# Autodesk Inventor assembly: 174376 FNC-32
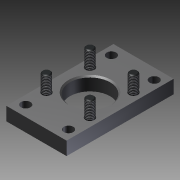
[picture p0: Inventor's stored thumbnail of the model, 180x180]
Saved by Autodesk Inventor 2011 SP1 (Build 150282100, 282)
## iProperties
Created: 2018-05-26
Part Number: 174376 FNC-32
Catalog Web Link: www.cadenas.de
Description: FNC-Flange mounting
Vendor: FESTO
Document SubType Name: Assembly
Designer: psAdmin
Manufacturer: FESTO
Mass: 221 g
Category: PARTsolutions
Company: FESTO
Title: 174376 FNC-32
Author: Cadenas PARTsolutions
Comments: Flange mounting
PSOL_IDENT_0: {$CADENAS_DATA\23d-libs\festo\parts\f\fnc\fnc_asmtab.prj},179 {VTYP=3D},{STYP=ASSTAB},{NB=174376 FNC
PSOL_IDENT_1: -32},{LINA=174376 FNC-32},{NN=FNC},{DATE=02.09.2015 15:05:29},{GEOMDATE=02.09.2015 15:05:29},{VERSIO
PSOL_IDENT_2: N=},{LINEID=10},{LINESUBID=-1},{WBVAR=}  {NB=174376 FNC-32},{LINA=174376 FNC-32},{KT=DUMMY},{TNR=174
PSOL_IDENT_3: 376},{TYP=FNC-32},{VERS=2},{D1=30.000},{D2=6.600},{D3=10.500},{E=45.000},{F=1.000},{FB=7.000},{MF=10
PSOL_IDENT_4: .000},{R=32.000},{T=5.000},{TF=64.000},{TG1=32.500},{UF=80.000},{CNSMASSEXACT=0.221},{ZZ=0},{DK=32},
PSOL_IDENT_5: {D6912D=6.000},{D6912L=18.000},{PPATH=assemblies/fnc_asmtpl.prj}
NN: FNC
NT: Flange mounting
NB: 174376 FNC-32
NBSYN: $TNR. $TYP.
LINA: 174376 FNC-32
TNR: 174376
TYP: FNC-32
D1: 30.000
D2: 6.600
D3: 10.500
E: 45.000
F: 1.000
FB: 7.000
MF: 10.000
R: 32.000
T: 5.000
TF: 64.000
TG1: 32.500
UF: 80.000
CNSMASSEXACT: 0.221
SUPPLIER: FESTO
ARTICLENO: 174376 FNC-32
BOMINFO: 174376 FNC-32
CREATOR: CADENAS GmbH
## Documents named in this file (3)
- p:\temp\worker_2\2692_1244\cad_41_02018052614572452943483192d056f_000000_00_00_000001\174376 FNC-32.iam
- p:\temp\worker_2\2692_1244\cad_41_02018052614572452943483192d056f_000000_00_00_000001\174376 FNC-32---(F).ipt
- p:\temp\worker_2\2692_1244\cad_41_02018052614572452943483192d056f_000000_00_00_000001\DIN-6912 - M6x18(F).ipt
## Components (5 placed, 2 different names)
1. 174376 FNC-32---(F):1 — FNC_Schraube_1_XY@1 <-> MONTAGE_XY@2, FNC_Schraube_1_Z@1 <-> MONTAGE_Z@2, FNC_Schraube_2_XY@1 <-> MONTAGE_XY@3, FNC_Schraube_2_Z@1 <-> MONTAGE_Z@3, FNC_Schraube_2_YZ@1 <-> MONTAGE_YZ@3, FNC_Schraube_3_XY@1 <-> MONTAGE_XY@4, FNC_Schraube_3_Z@1 <-> MONTAGE_Z@4, FNC_Schraube_3_YZ@1 <-> MONTAGE_YZ@4, FNC_Schraube_4_XY@1 <-> MONTAGE_XY@5, FNC_Schraube_4_Z@1 <-> MONTAGE_Z@5
2. DIN-6912 - M6x18(F):1 — FNC_Schraube_1_XY@1 <-> MONTAGE_XY@2, FNC_Schraube_1_Z@1 <-> MONTAGE_Z@2
3. DIN-6912 - M6x18(F):2 — FNC_Schraube_2_XY@1 <-> MONTAGE_XY@3, FNC_Schraube_2_Z@1 <-> MONTAGE_Z@3, FNC_Schraube_2_YZ@1 <-> MONTAGE_YZ@3
4. DIN-6912 - M6x18(F):3 — FNC_Schraube_3_XY@1 <-> MONTAGE_XY@4, FNC_Schraube_3_Z@1 <-> MONTAGE_Z@4, FNC_Schraube_3_YZ@1 <-> MONTAGE_YZ@4
5. DIN-6912 - M6x18(F):4 — FNC_Schraube_4_XY@1 <-> MONTAGE_XY@5, FNC_Schraube_4_Z@1 <-> MONTAGE_Z@5
## Relationships (10: Flush 4, Mate 4, Angle 2)
- FNC_Schraube_1_XY@1 <-> MONTAGE_XY@2 [Flush]: 174376 FNC-32---(F):1 ↔ DIN-6912 - M6x18(F):1
- FNC_Schraube_1_Z@1 <-> MONTAGE_Z@2 [Mate]: 174376 FNC-32---(F):1 ↔ DIN-6912 - M6x18(F):1
- FNC_Schraube_2_XY@1 <-> MONTAGE_XY@3 [Flush]: 174376 FNC-32---(F):1 ↔ DIN-6912 - M6x18(F):2
- FNC_Schraube_2_Z@1 <-> MONTAGE_Z@3 [Mate]: 174376 FNC-32---(F):1 ↔ DIN-6912 - M6x18(F):2
- FNC_Schraube_2_YZ@1 <-> MONTAGE_YZ@3 [Angle] (0 deg): 174376 FNC-32---(F):1 ↔ DIN-6912 - M6x18(F):2
- FNC_Schraube_3_XY@1 <-> MONTAGE_XY@4 [Flush]: 174376 FNC-32---(F):1 ↔ DIN-6912 - M6x18(F):3
- FNC_Schraube_3_Z@1 <-> MONTAGE_Z@4 [Mate]: 174376 FNC-32---(F):1 ↔ DIN-6912 - M6x18(F):3
- FNC_Schraube_3_YZ@1 <-> MONTAGE_YZ@4 [Angle] (0 deg): 174376 FNC-32---(F):1 ↔ DIN-6912 - M6x18(F):3
- FNC_Schraube_4_XY@1 <-> MONTAGE_XY@5 [Flush]: 174376 FNC-32---(F):1 ↔ DIN-6912 - M6x18(F):4
- FNC_Schraube_4_Z@1 <-> MONTAGE_Z@5 [Mate]: 174376 FNC-32---(F):1 ↔ DIN-6912 - M6x18(F):4
